# Autodesk Inventor assembly: wheel with sprocket
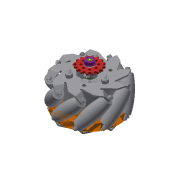
[picture p0: Inventor's stored thumbnail of the model, 180x180]
Saved by Autodesk Inventor 2019 (Build 230136000, 136)
## iProperties
Created: 2019-09-29
Part Number: wheel with sprocket
Document SubType Name: Assembly
Designer: ball
Author: ball
## Documents named in this file (6)
- C:\FTC\FTC8863CAD\2019 Robot\Mecanum Drive Train\wheel with sprocket.iam
- C:\FTC\FTC8863CAD\2019 Robot\Mecanum Drive Train\left wheel with clamping hub.iam
- C:\FTC\FTC8863CAD\Actobotics\615 parts\615102.ipt
- C:\FTC\FTC8863CAD\Actobotics\535 parts\535198.ipt
- C:\FTC\FTC8863CAD\Actobotics\633 parts\633104.ipt
- C:\FTC\FTC8863CAD\2019 Robot\Mecanum Drive Train\3_2 shaft.ipt
## Components (7 placed, 5 different names)
1. left wheel with clamping hub:1 [sub-assembly] — Mate:1, Mate:2, Mate:3, Mate:4, Mate:5, Mate:16, Mate:17, Mate:19
2. 615102:1 — Mate:1, Mate:2, Mate:3, Mate:7, Mate:13, Mate:14
3. 535198:1 — Mate:18, Mate:19
4. 535198:2 — Mate:7, Mate:15, Mate:20, Flush:1
5. 633104:1 — Mate:16, Mate:17, Mate:18
6. 633104:2 — Mate:13, Mate:14, Mate:15
7. 3_2 shaft:1 — Mate:20, Flush:1
## Relationships (15: Mate 14, Flush 1)
- Mate:1: left wheel with clamping hub:1 ↔ 615102:1
- Mate:2: left wheel with clamping hub:1 ↔ 615102:1
- Mate:3: left wheel with clamping hub:1 ↔ 615102:1
- Mate:4: left wheel with clamping hub:1
- Mate:5: left wheel with clamping hub:1
- Mate:7: 615102:1 ↔ 535198:2
- Mate:13: 615102:1 ↔ 633104:2
- Mate:14: 615102:1 ↔ 633104:2
- Mate:15: 535198:2 ↔ 633104:2
- Mate:16: left wheel with clamping hub:1 ↔ 633104:1
- Mate:17: left wheel with clamping hub:1 ↔ 633104:1
- Mate:18: 535198:1 ↔ 633104:1
- Mate:19: left wheel with clamping hub:1 ↔ 535198:1
- Mate:20: 535198:2 ↔ 3_2 shaft:1
- Flush:1: 535198:2 ↔ 3_2 shaft:1
